# Autodesk Inventor assembly: micro_usb_connector
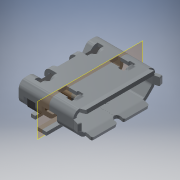
[picture p0: Inventor's stored thumbnail of the model, 180x180]
Saved by Autodesk Inventor 2017 (Build 210142000, 142)
## iProperties
Created: 2017-09-04
Part Number: micro_usb_connector
Document SubType Name: Assembly
Designer: intelsath
Sending System: Autodesk Translation Framework v6.1.1.50
Preprocessor: ST-DEVELOPER v16.13
Title: c:\worker\convert-fusion-jul-2017\tmp\job-1\1\output\files\e7196a44-a109-48ff-9976-57fbb18c6159\0f69fba3-69fe-4885-928e-7f0466b52a0b.stp
## Documents named in this file (5)
- C:\Users\intelsath\Documents\Inventor\Cryptowallet\micro_usb_connector.iam
- C:\Users\intelsath\Documents\Inventor\Cryptowallet\shield.ipt
- C:\Users\intelsath\Documents\Inventor\Cryptowallet\socket_housing.ipt
- C:\Users\intelsath\Documents\Inventor\Cryptowallet\socket_plate.ipt
- C:\Users\intelsath\Documents\Inventor\Cryptowallet\terminal.ipt
## Components (8 placed, 4 different names)
1. shield:1 — Mate:1, Mate:2, Angle:1
2. socket_housing:1
3. socket_plate:1
4. terminal:1
5. terminal:2
6. terminal:3
7. terminal:4
8. terminal:5
## Relationships (3: Mate 2, Angle 1)
- Mate:1: shield:1
- Mate:2: shield:1
- Angle:1 (0 deg): shield:1
